# Autodesk Inventor assembly: knuckle joint
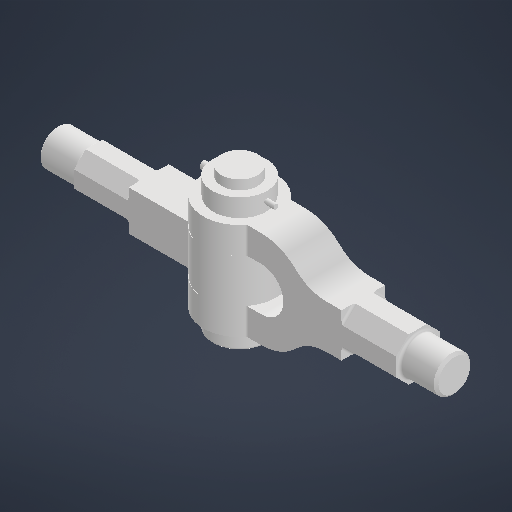
[picture p0: Inventor's stored thumbnail of the model, 512x512]
Saved by Autodesk Inventor 2026.3 (Build 303398000, 398)
## iProperties
Created: 2026-07-15
Part Number: knuckle joint
Document SubType Name: Assembly
Designer: User
Author: User
## Documents named in this file (6)
- C:\Users\User\Downloads\knuckle joint\knuckle joint.iam
- C:\Users\User\Downloads\knuckle joint\fork end.ipt
- C:\Users\User\Downloads\knuckle joint\eye end.ipt
- C:\Users\User\Downloads\knuckle joint\pin.ipt
- C:\Users\User\Downloads\knuckle joint\taper pin.ipt
- C:\Users\User\Downloads\knuckle joint\collor.ipt
## Components (5 placed, 5 different names)
1. fork end:1 — Flush:1, Mate:1, Mate:2, Mate:3, Mate:4, Mate:5, Mate:6, Tangent:1
2. eye end:1 — Mate:3, Mate:4, Mate:5, Mate:7
3. pin:1 — Mate:6, Mate:7, Mate:8
4. taper pin:1 — Mate:8, Tangent:1, Mate:9, Mate:10
5. collor:1 — Mate:9, Mate:10
## Relationships (12: Mate 10, Flush 1, Tangent 1)
- Flush:1: fork end:1
- Mate:1: fork end:1
- Mate:2: fork end:1
- Mate:3: fork end:1 ↔ eye end:1
- Mate:4: fork end:1 ↔ eye end:1
- Mate:5: fork end:1 ↔ eye end:1
- Mate:6: fork end:1 ↔ pin:1
- Mate:7: eye end:1 ↔ pin:1
- Mate:8: pin:1 ↔ taper pin:1
- Tangent:1 (-30 mm): fork end:1 ↔ taper pin:1
- Mate:9: taper pin:1 ↔ collor:1
- Mate:10 (-30 mm): taper pin:1 ↔ collor:1
